# Autodesk Inventor assembly: s-assy-driver
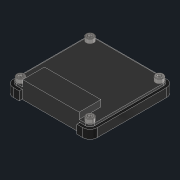
[picture p0: Inventor's stored thumbnail of the model, 180x180]
Saved by Autodesk Inventor 2022 (Build 260153000, 153)
## iProperties
Created: 2021-09-16
Part Number: s-assy-driver
Document SubType Name: Assembly
Designer: Yuta Kage
Author: Yuta Kage
## Documents named in this file (6)
- C:\Users\yuta0\Documents\GitHub\catchrobo_hardware\assy-robot\s-assy-driver.iam
- C:\Users\yuta0\Documents\GitHub\catchrobo_hardware\assy-robot\base47.ipt
- C:\Users\yuta0\Documents\GitHub\zebra_hardware\hardware\zebra_cad_v1.0\driver_ver1.0.ipt
- C:\Users\yuta0\Documents\GitHub\catchrobo_hardware\assy-robot\LBNR3.ipt
- C:\Users\yuta0\Documents\GitHub\catchrobo_hardware\assy-robot\CB3-6.ipt
- C:\Users\yuta0\Documents\GitHub\catchrobo_hardware\assy-robot\CB3-10.ipt
## Components (13 placed, 5 different names)
1. base47:1 — メイト:4, 角度:1, メイト:5, メイト:6, メイト:7, メイト:8, メイト:11, メイト:12
2. driver_ver1.0:1 — メイト:6, メイト:7, メイト:8, メイト:9, メイト:10
3. CB3-6:1 — メイト:9, メイト:10
4. LBNR3:1 — メイト:4, 角度:1, メイト:5
5. CB3-6:2
6. LBNR3:2
7. CB3-6:3
8. LBNR3:3
9. CB3-6:4
10. LBNR3:4
11. CB3-10:1 — メイト:11, メイト:12
12. CB3-10:2
13. CB3-10:3
## Component patterns: (4 elements, first: CB3-6:1 + LBNR3:1), (3 elements, first: CB3-10:1)
## Relationships (10: Mate 9, Angle 1)
- メイト:4 [Mate]: base47:1 ↔ LBNR3:1
- 角度:1 [Angle] (0 deg): base47:1 ↔ LBNR3:1
- メイト:5 [Mate]: base47:1 ↔ LBNR3:1
- メイト:6 [Mate]: base47:1 ↔ driver_ver1.0:1
- メイト:7 [Mate]: base47:1 ↔ driver_ver1.0:1
- メイト:8 [Mate]: base47:1 ↔ driver_ver1.0:1
- メイト:9 [Mate]: driver_ver1.0:1 ↔ CB3-6:1
- メイト:10 [Mate]: driver_ver1.0:1 ↔ CB3-6:1
- メイト:11 [Mate]: base47:1 ↔ CB3-10:1
- メイト:12 [Mate]: base47:1 ↔ CB3-10:1
